# Autodesk Inventor assembly: A2017_T2_07
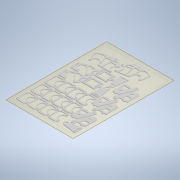
[picture p0: Inventor's stored thumbnail of the model, 180x180]
Saved by Autodesk Inventor 2020 (Build 240168000, 168)
## iProperties
Created: 2021-08-27
Part Number: A2017_T2_07
Document SubType Name: Assembly
Designer: Masato
Author: Masato
## Documents named in this file (7)
- C:\Inventor\SUSTAINA-OP\Cam\A2017_T2_07.iam
- C:\Inventor\SUSTAINA-OP\Cam\DisposableBoard.ipt
- C:\Inventor\SUSTAINA-OP\LowerBody\Ankle\Ankle_back_frame.ipt
- C:\Inventor\SUSTAINA-OP\LowerBody\Foot\Foot_front_frame.ipt
- C:\Inventor\SUSTAINA-OP\LowerBody\Leg_joint\Leg_joint_pitch_frame.ipt
- C:\Inventor\SUSTAINA-OP\LowerBody\Ankle\Ankle_side_frame.ipt
- C:\Inventor\SUSTAINA-OP\LowerBody\Knee\Knee_side_frame.ipt
## Components (26 placed, 6 different names)
1. DisposableBoard:1 — メイト:2, メイト:1, フラッシュ:1, フラッシュ:2, メイト:4, メイト:5, メイト:6, メイト:7, メイト:9, メイト:10, メイト:11, メイト:12, メイト:13, メイト:17, メイト:21, メイト:22, メイト:23, メイト:26, メイト:28, 正接:2, メイト:30, メイト:34, フラッシュ:7, メイト:35, 角度:1
2. Foot_front_frame:1 — メイト:17, メイト:21, フラッシュ:3, フラッシュ:4, 正接:1
3. Knee_side_frame:1 — メイト:28, メイト:29, 正接:2, 正接:4
4. Knee_side_frame:2 — メイト:34, フラッシュ:7, 正接:4
5. Foot_front_frame:2 — メイト:30, メイト:31, メイト:32, 正接:6
6. Foot_front_frame:4 — メイト:35, 正接:5, 角度:1, 正接:6
7. Ankle_back_frame:1 — メイト:4, メイト:9, メイト:10, メイト:14
8. Ankle_back_frame:2 — メイト:5, メイト:11, メイト:14, メイト:15
9. Ankle_back_frame:3 — メイト:6, メイト:12, メイト:15, メイト:16
10. Ankle_back_frame:4 — メイト:7, メイト:13, メイト:16, フラッシュ:3
11. Ankle_back_frame:5
12. Ankle_back_frame:6
13. Ankle_back_frame:7
14. Ankle_back_frame:8 — メイト:25
15. Ankle_back_frame:9 — フラッシュ:5, メイト:27
16. Ankle_back_frame:10
17. Ankle_back_frame:11
18. Ankle_back_frame:12 — メイト:31
19. Leg_joint_pitch_frame:1 — メイト:22, フラッシュ:4, 正接:1, メイト:24
20. Leg_joint_pitch_frame:2 — メイト:23, メイト:24, メイト:25
21. Leg_joint_pitch_frame:3
22. Leg_joint_pitch_frame:4 — メイト:32
23. Leg_joint_pitch_frame:5
24. Leg_joint_pitch_frame:6
25. Ankle_side_frame:1 — メイト:26, フラッシュ:5, メイト:27
26. Ankle_side_frame:2 — メイト:29, 正接:5
## Component patterns: (3 elements, first: Ankle_back_frame:1 + Ankle_back_frame:2 + Ankle_back_frame:3 + Ankle_back_frame:4), (3 elements, first: Leg_joint_pitch_frame:1 + Leg_joint_pitch_frame:2), (2 elements, first: Ankle_side_frame:1)
## Relationships (41: Mate 29, Flush 6, Tangent 5, Angle 1)
- メイト:2 [Mate]: DisposableBoard:1
- メイト:1 [Mate]: DisposableBoard:1
- フラッシュ:1 [Flush]: DisposableBoard:1
- フラッシュ:2 [Flush]: DisposableBoard:1
- メイト:4 [Mate]: DisposableBoard:1 ↔ Ankle_back_frame:1
- メイト:5 [Mate]: DisposableBoard:1 ↔ Ankle_back_frame:2
- メイト:6 [Mate]: DisposableBoard:1 ↔ Ankle_back_frame:3
- メイト:7 [Mate]: DisposableBoard:1 ↔ Ankle_back_frame:4
- メイト:9 [Mate] (3 mm): DisposableBoard:1 ↔ Ankle_back_frame:1
- メイト:10 [Mate] (3 mm): DisposableBoard:1 ↔ Ankle_back_frame:1
- メイト:11 [Mate] (3 mm): DisposableBoard:1 ↔ Ankle_back_frame:2
- メイト:12 [Mate] (3 mm): DisposableBoard:1 ↔ Ankle_back_frame:3
- メイト:13 [Mate] (3 mm): DisposableBoard:1 ↔ Ankle_back_frame:4
- メイト:14 [Mate] (2.5 mm): Ankle_back_frame:1 ↔ Ankle_back_frame:2
- メイト:15 [Mate] (2.5 mm): Ankle_back_frame:2 ↔ Ankle_back_frame:3
- メイト:16 [Mate] (2.5 mm): Ankle_back_frame:3 ↔ Ankle_back_frame:4
- メイト:17 [Mate]: DisposableBoard:1 ↔ Foot_front_frame:1
- メイト:21 [Mate] (3 mm): DisposableBoard:1 ↔ Foot_front_frame:1
- フラッシュ:3 [Flush]: Foot_front_frame:1 ↔ Ankle_back_frame:4
- メイト:22 [Mate]: DisposableBoard:1 ↔ Leg_joint_pitch_frame:1
- フラッシュ:4 [Flush]: Foot_front_frame:1 ↔ Leg_joint_pitch_frame:1
- 正接:1 [Tangent] (2.5 mm): Foot_front_frame:1 ↔ Leg_joint_pitch_frame:1
- メイト:23 [Mate]: DisposableBoard:1 ↔ Leg_joint_pitch_frame:2
- メイト:24 [Mate] (2.5 mm): Leg_joint_pitch_frame:1 ↔ Leg_joint_pitch_frame:2
- メイト:25 [Mate] (2.5 mm): Ankle_back_frame:8 ↔ Leg_joint_pitch_frame:2
- メイト:26 [Mate]: DisposableBoard:1 ↔ Ankle_side_frame:1
- フラッシュ:5 [Flush]: Ankle_back_frame:9 ↔ Ankle_side_frame:1
- メイト:27 [Mate] (2.5 mm): Ankle_back_frame:9 ↔ Ankle_side_frame:1
- メイト:28 [Mate]: DisposableBoard:1 ↔ Knee_side_frame:1
- メイト:29 [Mate] (2.5 mm): Knee_side_frame:1 ↔ Ankle_side_frame:2
- 正接:2 [Tangent] (2.5 mm): DisposableBoard:1 ↔ Knee_side_frame:1
- メイト:30 [Mate]: DisposableBoard:1 ↔ Foot_front_frame:2
- メイト:31 [Mate] (2.5 mm): Foot_front_frame:2 ↔ Ankle_back_frame:12
- メイト:32 [Mate] (3.5 mm): Foot_front_frame:2 ↔ Leg_joint_pitch_frame:4
- メイト:34 [Mate]: DisposableBoard:1 ↔ Knee_side_frame:2
- フラッシュ:7 [Flush] (2.5 mm): DisposableBoard:1 ↔ Knee_side_frame:2
- 正接:4 [Tangent] (2.5 mm): Knee_side_frame:1 ↔ Knee_side_frame:2
- メイト:35 [Mate]: DisposableBoard:1 ↔ Foot_front_frame:4
- 正接:5 [Tangent] (2.5 mm): Foot_front_frame:4 ↔ Ankle_side_frame:2
- 角度:1 [Angle] (0 deg): DisposableBoard:1 ↔ Foot_front_frame:4
- 正接:6 [Tangent] (2.5 mm): Foot_front_frame:2 ↔ Foot_front_frame:4
